# Autodesk Inventor assembly: AM14U3 Long Frame Half
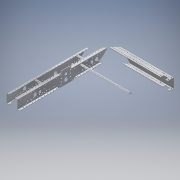
[picture p0: Inventor's stored thumbnail of the model, 180x180]
Saved by Autodesk Inventor 2016 (Build 200138000, 138)
## iProperties
Created: 2016-01-13
Part Number: AM14U3 Long Frame Half
Document SubType Name: Assembly
Designer: Douglas
Author: Douglas
Revision Number: ANY
## Documents named in this file (9)
- D:\SkyDrive\GitHub\2016-Robot-CAD\Inventor\Chassis\AM14U3 Long Frame Half.iam
- D:\SkyDrive\GitHub\2016-Robot-CAD\Inventor\Chassis\Churro 3375.ipt
- D:\SkyDrive\GitHub\2016-Robot-CAD\Inventor\Chassis\FHTS 0.25-20-0.75_FHTS 0.25-20-G-0.75-C.ipt
- D:\SkyDrive\GitHub\2016-Robot-CAD\Inventor\Chassis\Churro 16250.ipt
- D:\SkyDrive\GitHub\2016-Robot-CAD\Inventor\Chassis\10-32x0500_shcs_HX-SHCS 0.19-32x1.375x1-C.ipt
- D:\SkyDrive\GitHub\2016-Robot-CAD\Inventor\Chassis\10-32 Nylock Nut.ipt
- D:\SkyDrive\GitHub\2016-Robot-CAD\Inventor\Chassis\AM14U3 End Sheet Long.ipt
- D:\SkyDrive\GitHub\2016-Robot-CAD\Inventor\Chassis\AM14U3 Inside Sheet Rev2.ipt
- D:\SkyDrive\GitHub\2016-Robot-CAD\Inventor\Chassis\AM14U3 Outside Sheet Rev1_DefaultSM-FLAT-PATTERN.ipt
## Components (42 placed, 42 different names)
1. Churro 3375_80 — Mate:1, Mate:2, Mate:3, Mate:5
2. Churro 3375_81 — Mate:58, Mate:59, Mate:60, Mate:62
3. Churro 3375_82 — Mate:7, Mate:8, Mate:9, Mate:10
4. Churro 3375_83 — Mate:52, Mate:53, Mate:54, Mate:55
5. FHTS 0.25-20-0.75_FHTS 0.25-20-G-0.75-C_84 — Mate:60, Mate:61
6. FHTS 0.25-20-0.75_FHTS 0.25-20-G-0.75-C_85 — Mate:3, Mate:4
7. FHTS 0.25-20-0.75_FHTS 0.25-20-G-0.75-C_86 — Mate:9, Mate:12
8. FHTS 0.25-20-0.75_FHTS 0.25-20-G-0.75-C_87 — Mate:55, Mate:56
9. FHTS 0.25-20-0.75_FHTS 0.25-20-G-0.75-C_88 — Mate:62, Mate:63
10. FHTS 0.25-20-0.75_FHTS 0.25-20-G-0.75-C_89 — Mate:5, Mate:6
11. FHTS 0.25-20-0.75_FHTS 0.25-20-G-0.75-C_90 — Mate:54, Mate:57
12. FHTS 0.25-20-0.75_FHTS 0.25-20-G-0.75-C_91 — Mate:10, Mate:11
13. FHTS 0.25-20-0.75_FHTS 0.25-20-G-0.75-C_92
14. FHTS 0.25-20-0.75_FHTS 0.25-20-G-0.75-C_93
15. Churro 16250_94
16. 10-32x0500_shcs_HX-SHCS 0.19-32x1.375x1-C_95 — Mate:71, Mate:72, Mate:73
17. 10-32x0500_shcs_HX-SHCS 0.19-32x1.375x1-C_96 — Mate:77, Mate:78, Mate:79
18. 10-32x0500_shcs_HX-SHCS 0.19-32x1.375x1-C_97 — Mate:67, Mate:68, Mate:69
19. 10-32x0500_shcs_HX-SHCS 0.19-32x1.375x1-C_98 — Mate:75, Mate:76, Mate:80
20. 10-32x0500_shcs_HX-SHCS 0.19-32x1.375x1-C_99 — Mate:84, Mate:85, Mate:88
21. 10-32x0500_shcs_HX-SHCS 0.19-32x1.375x1-C_100 — Mate:83, Mate:86, Mate:87
22. 10-32x0500_shcs_HX-SHCS 0.19-32x1.375x1-C_101
23. 10-32x0500_shcs_HX-SHCS 0.19-32x1.375x1-C_102
24. 10-32x0500_shcs_HX-SHCS 0.19-32x1.375x1-C_103
25. 10-32x0500_shcs_HX-SHCS 0.19-32x1.375x1-C_104
26. 10-32x0500_shcs_HX-SHCS 0.19-32x1.375x1-C_105
27. 10-32x0500_shcs_HX-SHCS 0.19-32x1.375x1-C_106
28. 10-32 Nylock Nut_107
29. 10-32 Nylock Nut_108
30. 10-32 Nylock Nut_109
31. 10-32 Nylock Nut_110
32. 10-32 Nylock Nut_111
33. 10-32 Nylock Nut_112
34. 10-32 Nylock Nut_113 — Mate:69, Mate:70
35. 10-32 Nylock Nut_114 — Mate:80, Mate:81
36. 10-32 Nylock Nut_115 — Mate:73, Mate:74
37. 10-32 Nylock Nut_116 — Mate:79, Mate:82
38. 10-32 Nylock Nut_117 — Mate:88, Mate:90
39. 10-32 Nylock Nut_118 — Mate:87, Mate:89
40. AM14U3 End Sheet Long_135 — Mate:64, Mate:65, Mate:66, Mate:67, Mate:70, Mate:71, Mate:74, Mate:81, Mate:82, Mate:83, Mate:89, Mate:90
41. AM14U3 Inside Sheet Rev2_136 — Mate:1, Mate:2, Mate:4, Mate:7, Mate:8, Mate:12, Mate:52, Mate:56, Mate:58, Mate:61, Mate:64, Mate:75, Mate:76, Mate:77, Mate:78, Mate:84, Mate:85
42. AM14U3 Outside Sheet Rev1_DefaultSM-FLAT-PATTERN_137 — Mate:6, Mate:11, Mate:53, Mate:57, Mate:59, Mate:63, Mate:65, Mate:66, Mate:68, Mate:72, Mate:86
## Relationships (51: Mate 51)
- Mate:1: Churro 3375_80 ↔ AM14U3 Inside Sheet Rev2_136
- Mate:2: Churro 3375_80 ↔ AM14U3 Inside Sheet Rev2_136
- Mate:3: Churro 3375_80 ↔ FHTS 0.25-20-0.75_FHTS 0.25-20-G-0.75-C_85
- Mate:4: FHTS 0.25-20-0.75_FHTS 0.25-20-G-0.75-C_85 ↔ AM14U3 Inside Sheet Rev2_136
- Mate:5: Churro 3375_80 ↔ FHTS 0.25-20-0.75_FHTS 0.25-20-G-0.75-C_89
- Mate:6: FHTS 0.25-20-0.75_FHTS 0.25-20-G-0.75-C_89 ↔ AM14U3 Outside Sheet Rev1_DefaultSM-FLAT-PATTERN_137
- Mate:7: Churro 3375_82 ↔ AM14U3 Inside Sheet Rev2_136
- Mate:8: Churro 3375_82 ↔ AM14U3 Inside Sheet Rev2_136
- Mate:9: Churro 3375_82 ↔ FHTS 0.25-20-0.75_FHTS 0.25-20-G-0.75-C_86
- Mate:10: Churro 3375_82 ↔ FHTS 0.25-20-0.75_FHTS 0.25-20-G-0.75-C_91
- Mate:11: FHTS 0.25-20-0.75_FHTS 0.25-20-G-0.75-C_91 ↔ AM14U3 Outside Sheet Rev1_DefaultSM-FLAT-PATTERN_137
- Mate:12: FHTS 0.25-20-0.75_FHTS 0.25-20-G-0.75-C_86 ↔ AM14U3 Inside Sheet Rev2_136
- Mate:52: Churro 3375_83 ↔ AM14U3 Inside Sheet Rev2_136
- Mate:53: Churro 3375_83 ↔ AM14U3 Outside Sheet Rev1_DefaultSM-FLAT-PATTERN_137
- Mate:54: Churro 3375_83 ↔ FHTS 0.25-20-0.75_FHTS 0.25-20-G-0.75-C_90
- Mate:55: Churro 3375_83 ↔ FHTS 0.25-20-0.75_FHTS 0.25-20-G-0.75-C_87
- Mate:56: FHTS 0.25-20-0.75_FHTS 0.25-20-G-0.75-C_87 ↔ AM14U3 Inside Sheet Rev2_136
- Mate:57: FHTS 0.25-20-0.75_FHTS 0.25-20-G-0.75-C_90 ↔ AM14U3 Outside Sheet Rev1_DefaultSM-FLAT-PATTERN_137
- Mate:58: Churro 3375_81 ↔ AM14U3 Inside Sheet Rev2_136
- Mate:59: Churro 3375_81 ↔ AM14U3 Outside Sheet Rev1_DefaultSM-FLAT-PATTERN_137
- Mate:60: Churro 3375_81 ↔ FHTS 0.25-20-0.75_FHTS 0.25-20-G-0.75-C_84
- Mate:61: FHTS 0.25-20-0.75_FHTS 0.25-20-G-0.75-C_84 ↔ AM14U3 Inside Sheet Rev2_136
- Mate:62: Churro 3375_81 ↔ FHTS 0.25-20-0.75_FHTS 0.25-20-G-0.75-C_88
- Mate:63: FHTS 0.25-20-0.75_FHTS 0.25-20-G-0.75-C_88 ↔ AM14U3 Outside Sheet Rev1_DefaultSM-FLAT-PATTERN_137
- Mate:64: AM14U3 End Sheet Long_135 ↔ AM14U3 Inside Sheet Rev2_136
- Mate:65: AM14U3 End Sheet Long_135 ↔ AM14U3 Outside Sheet Rev1_DefaultSM-FLAT-PATTERN_137
- Mate:66: AM14U3 End Sheet Long_135 ↔ AM14U3 Outside Sheet Rev1_DefaultSM-FLAT-PATTERN_137
- Mate:67: 10-32x0500_shcs_HX-SHCS 0.19-32x1.375x1-C_97 ↔ AM14U3 End Sheet Long_135
- Mate:68: 10-32x0500_shcs_HX-SHCS 0.19-32x1.375x1-C_97 ↔ AM14U3 Outside Sheet Rev1_DefaultSM-FLAT-PATTERN_137
- Mate:69: 10-32x0500_shcs_HX-SHCS 0.19-32x1.375x1-C_97 ↔ 10-32 Nylock Nut_113
- Mate:70: 10-32 Nylock Nut_113 ↔ AM14U3 End Sheet Long_135
- Mate:71: 10-32x0500_shcs_HX-SHCS 0.19-32x1.375x1-C_95 ↔ AM14U3 End Sheet Long_135
- Mate:72: 10-32x0500_shcs_HX-SHCS 0.19-32x1.375x1-C_95 ↔ AM14U3 Outside Sheet Rev1_DefaultSM-FLAT-PATTERN_137
- Mate:73: 10-32x0500_shcs_HX-SHCS 0.19-32x1.375x1-C_95 ↔ 10-32 Nylock Nut_115
- Mate:74: 10-32 Nylock Nut_115 ↔ AM14U3 End Sheet Long_135
- Mate:75: 10-32x0500_shcs_HX-SHCS 0.19-32x1.375x1-C_98 ↔ AM14U3 Inside Sheet Rev2_136
- Mate:76: 10-32x0500_shcs_HX-SHCS 0.19-32x1.375x1-C_98 ↔ AM14U3 Inside Sheet Rev2_136
- Mate:77: 10-32x0500_shcs_HX-SHCS 0.19-32x1.375x1-C_96 ↔ AM14U3 Inside Sheet Rev2_136
- Mate:78: 10-32x0500_shcs_HX-SHCS 0.19-32x1.375x1-C_96 ↔ AM14U3 Inside Sheet Rev2_136
- Mate:79: 10-32x0500_shcs_HX-SHCS 0.19-32x1.375x1-C_96 ↔ 10-32 Nylock Nut_116
- Mate:80: 10-32x0500_shcs_HX-SHCS 0.19-32x1.375x1-C_98 ↔ 10-32 Nylock Nut_114
- Mate:81: 10-32 Nylock Nut_114 ↔ AM14U3 End Sheet Long_135
- Mate:82: 10-32 Nylock Nut_116 ↔ AM14U3 End Sheet Long_135
- Mate:83: 10-32x0500_shcs_HX-SHCS 0.19-32x1.375x1-C_100 ↔ AM14U3 End Sheet Long_135
- Mate:84: 10-32x0500_shcs_HX-SHCS 0.19-32x1.375x1-C_99 ↔ AM14U3 Inside Sheet Rev2_136
- Mate:85: 10-32x0500_shcs_HX-SHCS 0.19-32x1.375x1-C_99 ↔ AM14U3 Inside Sheet Rev2_136
- Mate:86: 10-32x0500_shcs_HX-SHCS 0.19-32x1.375x1-C_100 ↔ AM14U3 Outside Sheet Rev1_DefaultSM-FLAT-PATTERN_137
- Mate:87: 10-32x0500_shcs_HX-SHCS 0.19-32x1.375x1-C_100 ↔ 10-32 Nylock Nut_118
- Mate:88: 10-32x0500_shcs_HX-SHCS 0.19-32x1.375x1-C_99 ↔ 10-32 Nylock Nut_117
- Mate:89: 10-32 Nylock Nut_118 ↔ AM14U3 End Sheet Long_135
- Mate:90: 10-32 Nylock Nut_117 ↔ AM14U3 End Sheet Long_135
